# Autodesk Inventor assembly: Lift Assembly Right
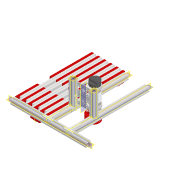
[picture p0: Inventor's stored thumbnail of the model, 180x180]
Saved by Autodesk Inventor 2020 (Build 240168000, 168)
## iProperties
Created: 2019-12-26
Part Number: Lift Assembly Right
Document SubType Name: Assembly
Designer: ball
Author: ball
## Documents named in this file (12)
- C:\FTC\FTC8863CAD\2019 Robot\Delivery\Lift Right\Lift Assembly Right.iam
- C:\FTC\FTC8863CAD\2019 Robot\Delivery\Lift Right\SAR330  x 5 + couplers right.iam
- C:\FTC\FTC8863CAD\Actobotics\565 parts\565046.ipt
- C:\FTC\FTC8863CAD\Actobotics\585 parts\585075.ipt
- C:\FTC\FTC8863CAD\Actobotics\565 parts\xrail_3.5in.ipt
- C:\FTC\FTC8863CAD\Actobotics\555 parts\555116 assembly.ipt
- C:\FTC\FTC8863CAD\Actobotics\585 parts\585721.ipt
- C:\FTC\FTC8863CAD\2019 Robot\Delivery\spool double 2 in diameter.iam
- C:\FTC\FTC8863CAD\Andymark\am-2964a Neverest Classic 40.ipt
- C:\FTC\FTC8863CAD\2019 Robot\Delivery\Lift Right\Limit switch top + mount right.iam
- C:\FTC\FTC8863CAD\StepLibraries\Screws\M3 x 25 HEX HEAD CAP SCREW.ipt
- C:\FTC\FTC8863CAD\2019 Robot\Delivery\Lift Right\Limit switch bottom + mount right.iam
## Components (20 placed, 11 different names)
1. SAR330  x 5 + couplers right:1 [sub-assembly] — Mate:8, Flush:2, Flush:3, Mate:9, Flush:4, Mate:18, Mate:25, Mate:26, Mate:48, Mate:49, Flush:10, Mate:51, Mate:53, Flush:11
2. 565046:1 — Mate:8, Flush:2, Flush:3, Mate:10, Mate:11, Mate:12, Mate:13, Mate:14, Flush:7, Mate:54, Mate:55
3. 585075:2
4. 565046:2 — Mate:11, Mate:12, Flush:6, Mate:16, Mate:24, Flush:9, Mate:31
5. 585075:4 — Mate:9, Mate:10, Flush:4
6. xrail_3.5in:2 — Mate:16, Flush:7, Flush:8, Mate:24, Mate:28, Mate:29, Symmetry:1, Mate:30, Mate:38
7. 585075:5 — Mate:19, Mate:26, Mate:27
8. 585075:6 — Mate:13, Mate:14, Flush:6
9. xrail_3.5in:3 — Mate:18, Flush:8, Mate:19, Mate:25, Mate:27, Symmetry:1, Mate:32, Mate:33, Mate:35
10. 585075:8 — Flush:9, Mate:28, Mate:29
11. 585721:1 — Mate:30, Mate:31, Mate:32, Mate:34, Mate:36, Mate:39, Mate:40
12. 585721:2 — Mate:33, Mate:34, Mate:35, Mate:38, Mate:41, Mate:42, Mate:43
13. 555116 assembly:3 — Mate:36, Mate:39, Mate:40, Mate:46
14. 555116 assembly:4 — Mate:41, Mate:42, Mate:43, Mate:47
15. spool double 2 in diameter:1 [sub-assembly]
16. am-2964a Neverest Classic 40:1 — Mate:46, Mate:47
17. Limit switch top + mount right:1 [sub-assembly] — Mate:48, Mate:49, Flush:10, Mate:50, Mate:52
18. M3 x 25 HEX HEAD CAP SCREW:1 — Mate:50, Mate:51
19. M3 x 25 HEX HEAD CAP SCREW:2 — Mate:52, Mate:53
20. Limit switch bottom + mount right:1 [sub-assembly] — Mate:54, Mate:55, Flush:11
## Relationships (53: Mate 43, Flush 9, Symmetry 1)
- [Mate]: 565046:1 ↔ 585075:2
- [Mate]: 565046:1 ↔ 585075:2
- Mate:8: SAR330  x 5 + couplers right:1 ↔ 565046:1
- Flush:2: SAR330  x 5 + couplers right:1 ↔ 565046:1
- Flush:3: SAR330  x 5 + couplers right:1 ↔ 565046:1
- Mate:9: SAR330  x 5 + couplers right:1 ↔ 585075:4
- Mate:10: 565046:1 ↔ 585075:4
- Flush:4: SAR330  x 5 + couplers right:1 ↔ 585075:4
- Mate:11: 565046:1 ↔ 565046:2
- Mate:12: 565046:1 ↔ 565046:2
- Mate:13: 565046:1 ↔ 585075:6
- Mate:14: 565046:1 ↔ 585075:6
- Flush:6: 565046:2 ↔ 585075:6
- Mate:16: 565046:2 ↔ xrail_3.5in:2
- Flush:7 (-100.2792 mm): 565046:1 ↔ xrail_3.5in:2
- Mate:18: SAR330  x 5 + couplers right:1 ↔ xrail_3.5in:3
- Flush:8: xrail_3.5in:2 ↔ xrail_3.5in:3
- Mate:19: 585075:5 ↔ xrail_3.5in:3
- Mate:24: 565046:2 ↔ xrail_3.5in:2
- Mate:25: SAR330  x 5 + couplers right:1 ↔ xrail_3.5in:3
- Mate:26: SAR330  x 5 + couplers right:1 ↔ 585075:5
- Mate:27: 585075:5 ↔ xrail_3.5in:3
- Flush:9: 565046:2 ↔ 585075:8
- Mate:28: xrail_3.5in:2 ↔ 585075:8
- Mate:29: xrail_3.5in:2 ↔ 585075:8
- Symmetry:1: xrail_3.5in:2 ↔ xrail_3.5in:3
- Mate:30: xrail_3.5in:2 ↔ 585721:1
- Mate:31: 565046:2 ↔ 585721:1
- Mate:32: xrail_3.5in:3 ↔ 585721:1
- Mate:33: xrail_3.5in:3 ↔ 585721:2
- Mate:34: 585721:1 ↔ 585721:2
- Mate:35: xrail_3.5in:3 ↔ 585721:2
- Mate:36: 585721:1 ↔ 555116 assembly:3
- Mate:38: xrail_3.5in:2 ↔ 585721:2
- Mate:39: 585721:1 ↔ 555116 assembly:3
- Mate:40: 585721:1 ↔ 555116 assembly:3
- Mate:41: 585721:2 ↔ 555116 assembly:4
- Mate:42: 585721:2 ↔ 555116 assembly:4
- Mate:43: 585721:2 ↔ 555116 assembly:4
- [Mate]: spool double 2 in diameter:1 ↔ am-2964a Neverest Classic 40:1
- [Mate]: spool double 2 in diameter:1 ↔ am-2964a Neverest Classic 40:1
- Mate:46: 555116 assembly:3 ↔ am-2964a Neverest Classic 40:1
- Mate:47: 555116 assembly:4 ↔ am-2964a Neverest Classic 40:1
- Mate:48: SAR330  x 5 + couplers right:1 ↔ Limit switch top + mount right:1
- Mate:49: SAR330  x 5 + couplers right:1 ↔ Limit switch top + mount right:1
- Flush:10 (2.54 mm): SAR330  x 5 + couplers right:1 ↔ Limit switch top + mount right:1
- Mate:50: Limit switch top + mount right:1 ↔ M3 x 25 HEX HEAD CAP SCREW:1
- Mate:51: SAR330  x 5 + couplers right:1 ↔ M3 x 25 HEX HEAD CAP SCREW:1
- Mate:52: Limit switch top + mount right:1 ↔ M3 x 25 HEX HEAD CAP SCREW:2
- Mate:53: SAR330  x 5 + couplers right:1 ↔ M3 x 25 HEX HEAD CAP SCREW:2
- Mate:54: 565046:1 ↔ Limit switch bottom + mount right:1
- Mate:55: 565046:1 ↔ Limit switch bottom + mount right:1
- Flush:11: SAR330  x 5 + couplers right:1 ↔ Limit switch bottom + mount right:1
